# Autodesk Inventor assembly: CasaJugueteAPM
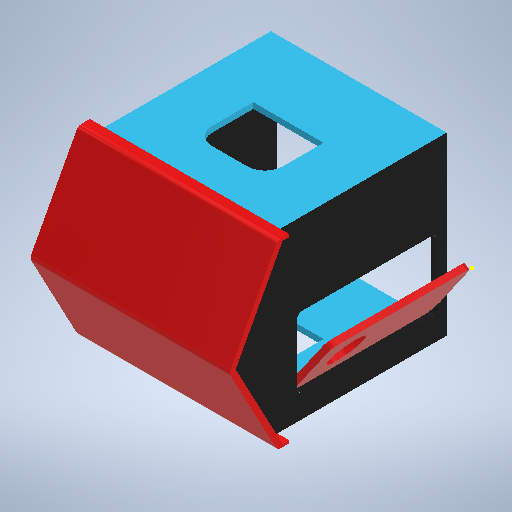
[picture p0: Inventor's stored thumbnail of the model, 512x512]
Saved by Autodesk Inventor 2025.2 (Build 292293000, 293)
## iProperties
Created: 2024-11-26
Part Number: CasaJugueteAPM
Document SubType Name: Assembly
Designer: usuario
Author: usuario
## Documents named in this file (3)
- C:\Users\usuario\Desktop\APM\ModeladosAPM\CasaJugueteAPM.iam
- C:\Users\usuario\Desktop\APM\ModeladosAPM\CasaJugueteAPM.ipt
- C:\Users\usuario\Desktop\APM\ModeladosAPM\Puerta.ipt
## Components (2 placed, 2 different names)
1. CasaJugueteAPM:1 — Coincidencia:1, Coincidencia:2
2. Puerta:1 — Coincidencia:1, Coincidencia:2
## Relationships (2: Mate 2)
- Coincidencia:1 [Mate]: CasaJugueteAPM:1 ↔ Puerta:1
- Coincidencia:2 [Mate]: CasaJugueteAPM:1 ↔ Puerta:1
